# Autodesk Inventor assembly: Robot
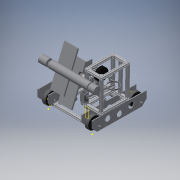
[picture p0: Inventor's stored thumbnail of the model, 180x180]
Saved by Autodesk Inventor 2017 (Build 210142000, 142)
## iProperties
Created: 2016-10-08
Part Number: Robot
Document SubType Name: Assembly
Designer: RoboticsUser
Author: RoboticsUser
## Documents named in this file (7)
- C:\Robotics\CAD\2016-17_CAD\Robot - CAD.iam
- C:\Robotics\CAD\COTSParts\Bosch Extrusion\Bosch 20x20 9 in - Copy.ipt
- C:\Robotics\CAD\2016-17_CAD\WheelAssemblyLeft.iam
- C:\Robotics\CAD\COTSParts\Bosch Extrusion\Bosch 20x20 9 real.ipt
- C:\Robotics\CAD\2016-17_CAD\CollectorHolderAssembly.iam
- C:\Robotics\CAD\2016-17_CAD\UpProto.ipt
- C:\Robotics\CAD\2016-17_CAD\ParticleLauncher2.0.iam
## Components (10 placed, 6 different names)
1. Bosch 20x20 9 in - Copy:1 — Flush:150, Mate:248, Flush:151, Flush:152, Mate:251, Flush:156, Flush:157, Mate:252, Flush:158, Mate:254, Flush:161, Mate:269
2. Bosch 20x20 9 in - Copy:2 — Mate:249, Flush:153, Flush:154, Mate:250, Flush:155, Flush:159, Mate:253, Flush:160
3. WheelAssemblyLeft:1 [sub-assembly] — Flush:154, Mate:250, Flush:155, Mate:253, Flush:160, Flush:162, Mate:268, Mate:270, Flush:174, Mate:276, Flush:175, Flush:176
4. WheelAssemblyLeft:2 [sub-assembly] — Flush:150, Mate:252, Flush:158, Mate:254, Flush:161, Flush:163, Mate:271, Mate:272, Mate:274, Mate:275, Flush:173
5. Bosch 20x20 9 real:1 — Mate:251, Flush:156, Flush:157, Mate:257
6. Bosch 20x20 9 real:2 — Mate:248, Flush:151, Flush:152, Mate:249, Flush:153, Flush:159, Flush:162, Flush:163
7. CollectorHolderAssembly:1 [sub-assembly] — Mate:273, Mate:274, Mate:275, Flush:173, Flush:174
8. UpProto:1 — Flush:171, Mate:267, Mate:268, Mate:270, Mate:271, Mate:273
9. UpProto:2 — Mate:257, Flush:171, Mate:267, Mate:269, Mate:272
10. ParticleLauncher2.0:1 [sub-assembly] — Mate:276, Flush:175, Flush:176
## Relationships (37: Flush 19, Mate 18)
- Flush:150: Bosch 20x20 9 in - Copy:1 ↔ WheelAssemblyLeft:2
- Mate:248: Bosch 20x20 9 in - Copy:1 ↔ Bosch 20x20 9 real:2
- Flush:151: Bosch 20x20 9 in - Copy:1 ↔ Bosch 20x20 9 real:2
- Flush:152: Bosch 20x20 9 in - Copy:1 ↔ Bosch 20x20 9 real:2
- Mate:249: Bosch 20x20 9 in - Copy:2 ↔ Bosch 20x20 9 real:2
- Flush:153: Bosch 20x20 9 in - Copy:2 ↔ Bosch 20x20 9 real:2
- Flush:154: Bosch 20x20 9 in - Copy:2 ↔ WheelAssemblyLeft:1
- Mate:250: Bosch 20x20 9 in - Copy:2 ↔ WheelAssemblyLeft:1
- Flush:155 (-38.1 mm): Bosch 20x20 9 in - Copy:2 ↔ WheelAssemblyLeft:1
- Mate:251: Bosch 20x20 9 in - Copy:1 ↔ Bosch 20x20 9 real:1
- Flush:156: Bosch 20x20 9 in - Copy:1 ↔ Bosch 20x20 9 real:1
- Flush:157: Bosch 20x20 9 in - Copy:1 ↔ Bosch 20x20 9 real:1
- Mate:252: Bosch 20x20 9 in - Copy:1 ↔ WheelAssemblyLeft:2
- Flush:158 (38.1 mm): Bosch 20x20 9 in - Copy:1 ↔ WheelAssemblyLeft:2
- Flush:159: Bosch 20x20 9 in - Copy:2 ↔ Bosch 20x20 9 real:2
- Mate:253: Bosch 20x20 9 in - Copy:2 ↔ WheelAssemblyLeft:1
- Mate:254: Bosch 20x20 9 in - Copy:1 ↔ WheelAssemblyLeft:2
- Flush:160: Bosch 20x20 9 in - Copy:2 ↔ WheelAssemblyLeft:1
- Flush:161: Bosch 20x20 9 in - Copy:1 ↔ WheelAssemblyLeft:2
- Flush:162 (38.1 mm): WheelAssemblyLeft:1 ↔ Bosch 20x20 9 real:2
- Flush:163 (38.1 mm): WheelAssemblyLeft:2 ↔ Bosch 20x20 9 real:2
- Mate:257: Bosch 20x20 9 real:1 ↔ UpProto:2
- Flush:171: UpProto:1 ↔ UpProto:2
- Mate:267 (95.25 mm): UpProto:1 ↔ UpProto:2
- Mate:268 (423.6974 mm): WheelAssemblyLeft:1 ↔ UpProto:1
- Mate:269 (-28.0924 mm): Bosch 20x20 9 in - Copy:1 ↔ UpProto:2
- Mate:270: WheelAssemblyLeft:1 ↔ UpProto:1
- Mate:271 (336.55 mm): WheelAssemblyLeft:2 ↔ UpProto:1
- Mate:272 (10.414 mm): WheelAssemblyLeft:2 ↔ UpProto:2
- Mate:273: CollectorHolderAssembly:1 ↔ UpProto:1
- Mate:274: WheelAssemblyLeft:2 ↔ CollectorHolderAssembly:1
- Mate:275: WheelAssemblyLeft:2 ↔ CollectorHolderAssembly:1
- Flush:173: WheelAssemblyLeft:2 ↔ CollectorHolderAssembly:1
- Flush:174 (128.905 mm): WheelAssemblyLeft:1 ↔ CollectorHolderAssembly:1
- Mate:276: WheelAssemblyLeft:1 ↔ ParticleLauncher2.0:1
- Flush:175: WheelAssemblyLeft:1 ↔ ParticleLauncher2.0:1
- Flush:176 (69.85 mm): WheelAssemblyLeft:1 ↔ ParticleLauncher2.0:1
